# Autodesk Inventor assembly: left wheel
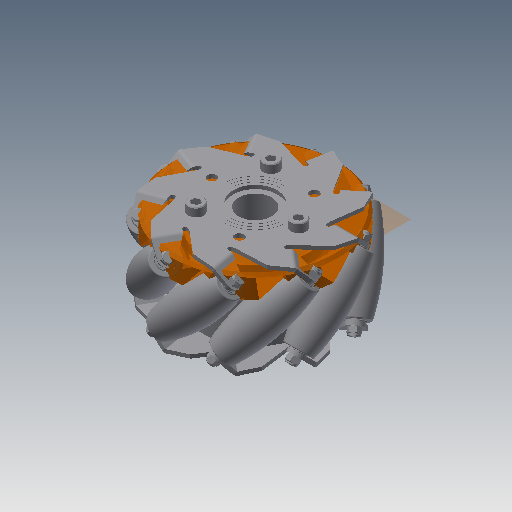
[picture p0: Inventor's stored thumbnail of the model, 512x512]
Saved by Autodesk Inventor 2020 (Build 240168000, 168)
## iProperties
Created: 2019-09-27
Part Number: left wheel
Document SubType Name: Assembly
Designer: ball
Author: ball
## Documents named in this file (4)
- C:\FTC\FTC8863CAD\2019 Robot\Mecanum Drive Train\left wheel.iam
- C:\FTC\FTC8863CAD\StepLibraries\Nuts\M5 NYLON-INSERT LOCKNUT.ipt
- C:\FTC\FTC8863CAD\Nexus-Wheels-STP\100mm Aluminum Mecanum wheels.ipt
- C:\FTC\FTC8863CAD\StepLibraries\Screws\M5 x 55 SOCKET HEAD CAP SCREW.ipt
## Components (7 placed, 3 different names)
1. M5 x 55 SOCKET HEAD CAP SCREW:1
2. M5 NYLON-INSERT LOCKNUT:1 — Mate:7
3. 100mm Aluminum Mecanum wheels:1 — Mate:7, Mate:8, Mate:9
4. M5 x 55 SOCKET HEAD CAP SCREW:2
5. M5 x 55 SOCKET HEAD CAP SCREW:3
6. M5 NYLON-INSERT LOCKNUT:2 — Mate:8
7. M5 NYLON-INSERT LOCKNUT:3 — Mate:9
## Relationships (12: Mate 12)
- [Mate]: M5 x 55 SOCKET HEAD CAP SCREW:1 ↔ 100mm Aluminum Mecanum wheels:1
- [Mate]: M5 x 55 SOCKET HEAD CAP SCREW:1 ↔ 100mm Aluminum Mecanum wheels:1
- [Mate]: 100mm Aluminum Mecanum wheels:1 ↔ M5 x 55 SOCKET HEAD CAP SCREW:3
- [Mate]: 100mm Aluminum Mecanum wheels:1 ↔ M5 x 55 SOCKET HEAD CAP SCREW:2
- [Mate]: 100mm Aluminum Mecanum wheels:1 ↔ M5 x 55 SOCKET HEAD CAP SCREW:2
- [Mate]: 100mm Aluminum Mecanum wheels:1 ↔ M5 x 55 SOCKET HEAD CAP SCREW:3
- Mate:7: M5 NYLON-INSERT LOCKNUT:1 ↔ 100mm Aluminum Mecanum wheels:1
- Mate:8: 100mm Aluminum Mecanum wheels:1 ↔ M5 NYLON-INSERT LOCKNUT:2
- Mate:9: 100mm Aluminum Mecanum wheels:1 ↔ M5 NYLON-INSERT LOCKNUT:3
- [Mate]: M5 x 55 SOCKET HEAD CAP SCREW:3 ↔ M5 NYLON-INSERT LOCKNUT:2
- [Mate]: M5 x 55 SOCKET HEAD CAP SCREW:1 ↔ M5 NYLON-INSERT LOCKNUT:3
- [Mate]: M5 NYLON-INSERT LOCKNUT:1 ↔ M5 x 55 SOCKET HEAD CAP SCREW:2
